# Autodesk Inventor assembly: rev1 base large wall
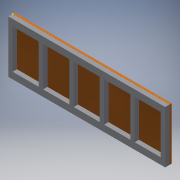
[picture p0: Inventor's stored thumbnail of the model, 180x180]
Saved by Autodesk Inventor 2017 (Build 210142000, 142)
## iProperties
Created: 2019-05-04
Part Number: rev1 base large wall
Document SubType Name: Assembly
Designer: Roman
Author: Roman
## Documents named in this file (4)
- C:\Users\Roman\Documents\CAD\enclosure rev1\rev2 base\rev1 large wall\rev1 base large wall.iam
- C:\Users\Roman\Documents\CAD\enclosure rev1\rev2 base\rev1 large wall\rev1 base large wall backplane.ipt
- C:\Users\Roman\Documents\CAD\enclosure rev1\rev2 base\rev1 large wall\rev1 base large wall h stud.ipt
- C:\Users\Roman\Documents\CAD\enclosure rev1\rev2 base\rev1 large wall\rev1 base large wall v stud.ipt
## Components (15 placed, 3 different names)
1. rev1 base large wall backplane:1 — Mate:1, Mate:2, Flush:1, Flush:2, Flush:3, Flush:4, Mate:4, Flush:5
2. rev1 base large wall h stud:1 — Mate:1, Flush:1, Flush:2, Mate:3
3. rev1 base large wall h stud:2 — Mate:2, Flush:3, Flush:4
4. rev1 base large wall v stud:1 — Mate:3, Mate:4, Flush:5
5. rev1 base large wall v stud:2
6. rev1 base large wall v stud:3
7. rev1 base large wall v stud:4
8. rev1 base large wall v stud:5
9. rev1 base large wall v stud:6
10. rev1 base large wall v stud:7
11. rev1 base large wall v stud:8
12. rev1 base large wall v stud:9
13. rev1 base large wall v stud:10
14. rev1 base large wall v stud:11
15. rev1 base large wall v stud:12
## Component patterns: (12 elements, first: rev1 base large wall v stud:1)
## Relationships (9: Flush 5, Mate 4)
- Mate:1: rev1 base large wall backplane:1 ↔ rev1 base large wall h stud:1
- Mate:2: rev1 base large wall backplane:1 ↔ rev1 base large wall h stud:2
- Flush:1: rev1 base large wall backplane:1 ↔ rev1 base large wall h stud:1
- Flush:2: rev1 base large wall backplane:1 ↔ rev1 base large wall h stud:1
- Flush:3: rev1 base large wall backplane:1 ↔ rev1 base large wall h stud:2
- Flush:4: rev1 base large wall backplane:1 ↔ rev1 base large wall h stud:2
- Mate:3: rev1 base large wall h stud:1 ↔ rev1 base large wall v stud:1
- Mate:4: rev1 base large wall backplane:1 ↔ rev1 base large wall v stud:1
- Flush:5: rev1 base large wall backplane:1 ↔ rev1 base large wall v stud:1
